# Autodesk Inventor assembly: Remastered_Overall_Shooting_Mechanism2
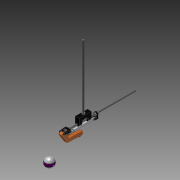
[picture p0: Inventor's stored thumbnail of the model, 180x180]
Saved by Autodesk Inventor 2015 (Build 190159000, 159)
## iProperties
Created: 2017-03-28
Part Number: Remastered_Overall_Shooting_Mechanism2
Document SubType Name: Assembly
Designer: Guy
Author: Guy
## Documents named in this file (11)
- C:\Users\Guy\Documents\Fourth Year\Capstone\git\Capstone-Project\doc\CAD\SM2\Remastered_Overall_Shooting_Mechanism2.iam
- C:\Users\Guy\Documents\Fourth Year\Capstone\git\Capstone-Project\doc\CAD\SM2\1-2in_eebase_connector.ipt
- C:\Users\Guy\Documents\Fourth Year\Capstone\git\Capstone-Project\doc\CAD\SM2\hinge_for_swing.ipt
- C:\Users\Guy\Documents\Fourth Year\Capstone\git\Capstone-Project\doc\CAD\SM2\Piston_Holder.ipt
- C:\Users\Guy\Documents\Fourth Year\Capstone\git\Capstone-Project\doc\CAD\SM2\piston_internal_rod.ipt
- C:\Users\Guy\Documents\Fourth Year\Capstone\git\Capstone-Project\doc\CAD\SM2\piston_rod_connector.ipt
- C:\Users\Guy\Documents\Fourth Year\Capstone\git\Capstone-Project\doc\CAD\SM2\Small_piston.ipt
- C:\Users\Guy\Documents\Fourth Year\Capstone\git\Capstone-Project\doc\CAD\SM2\swing_con2.ipt
- C:\Users\Guy\Documents\Fourth Year\Capstone\git\Capstone-Project\doc\CAD\LowLevel_Rev2\Pool_Ball_Stripe.ipt
- C:\Users\Guy\Documents\Fourth Year\Capstone\git\Capstone-Project\doc\CAD\SM2\EE_base_connection.ipt
- C:\Users\Guy\Documents\Fourth Year\Capstone\git\Capstone-Project\doc\CAD\ShootingMechanism\ThreadBarNut.ipt
## Components (16 placed, 10 different names)
1. 1-2in_eebase_connector:1 — Flush:1, Mate:1, Mate:4, Angle:1, Angle:2, Mate:15, Angle:3, Mate:21, Mate:22, Mate:25, Mate:26
2. hinge_for_swing:1 — Flush:1, Mate:1, Angle:1, Mate:7, Mate:12, Mate:13, Mate:27, Mate:28
3. Piston_Holder:1 — Mate:4, Mate:5, Mate:6, Angle:2, Mate:7, Mate:23, Mate:24
4. piston_internal_rod:1 — Mate:2, Mate:3, Flush:2
5. piston_rod_connector:1 — Mate:3, Flush:2, Mate:11, Mate:14
6. Small_piston:1 — Mate:2, Mate:5, Mate:6, Mate:11
7. swing_con2:1 — Mate:12, Mate:13, Mate:14
8. Pool_Ball_Stripe:2
9. EE_base_connection:1 — Mate:15, Mate:16, Angle:3, Mate:18, Mate:20
10. 1-2in_eebase_connector:2 — Mate:16, Mate:17, Mate:19, Flush:3
11. ThreadBarNut:1 — Mate:17, Mate:18
12. ThreadBarNut:2 — Mate:19, Mate:20, Flush:3
13. ThreadBarNut:3 — Mate:26, Mate:28
14. ThreadBarNut:4 — Mate:25, Mate:27
15. ThreadBarNut:5 — Mate:21, Mate:24
16. ThreadBarNut:6 — Mate:22, Mate:23
## Relationships (31: Mate 25, Flush 3, Angle 3)
- Flush:1: 1-2in_eebase_connector:1 ↔ hinge_for_swing:1
- Mate:1: 1-2in_eebase_connector:1 ↔ hinge_for_swing:1
- Mate:2: piston_internal_rod:1 ↔ Small_piston:1
- Mate:3: piston_internal_rod:1 ↔ piston_rod_connector:1
- Flush:2: piston_internal_rod:1 ↔ piston_rod_connector:1
- Mate:4: 1-2in_eebase_connector:1 ↔ Piston_Holder:1
- Mate:5: Piston_Holder:1 ↔ Small_piston:1
- Mate:6 (1 mm): Piston_Holder:1 ↔ Small_piston:1
- Angle:1 (0 deg): 1-2in_eebase_connector:1 ↔ hinge_for_swing:1
- Angle:2 (0 deg): 1-2in_eebase_connector:1 ↔ Piston_Holder:1
- Mate:7 (175 mm): hinge_for_swing:1 ↔ Piston_Holder:1
- Mate:11 (3 mm): piston_rod_connector:1 ↔ Small_piston:1
- Mate:12: hinge_for_swing:1 ↔ swing_con2:1
- Mate:13 (0.5 mm): hinge_for_swing:1 ↔ swing_con2:1
- Mate:14: piston_rod_connector:1 ↔ swing_con2:1
- Mate:15: 1-2in_eebase_connector:1 ↔ EE_base_connection:1
- Mate:16: EE_base_connection:1 ↔ 1-2in_eebase_connector:2
- Angle:3 (0 deg): 1-2in_eebase_connector:1 ↔ EE_base_connection:1
- Mate:17: 1-2in_eebase_connector:2 ↔ ThreadBarNut:1
- Mate:18: EE_base_connection:1 ↔ ThreadBarNut:1
- Mate:19: 1-2in_eebase_connector:2 ↔ ThreadBarNut:2
- Mate:20: EE_base_connection:1 ↔ ThreadBarNut:2
- Flush:3 (-5 mm): 1-2in_eebase_connector:2 ↔ ThreadBarNut:2
- Mate:21: 1-2in_eebase_connector:1 ↔ ThreadBarNut:5
- Mate:22: 1-2in_eebase_connector:1 ↔ ThreadBarNut:6
- Mate:23: Piston_Holder:1 ↔ ThreadBarNut:6
- Mate:24: Piston_Holder:1 ↔ ThreadBarNut:5
- Mate:25: 1-2in_eebase_connector:1 ↔ ThreadBarNut:4
- Mate:26: 1-2in_eebase_connector:1 ↔ ThreadBarNut:3
- Mate:27: hinge_for_swing:1 ↔ ThreadBarNut:4
- Mate:28: hinge_for_swing:1 ↔ ThreadBarNut:3
